# Autodesk Inventor assembly: Full Scale Assembly
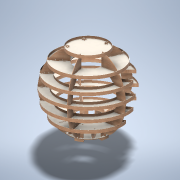
[picture p0: Inventor's stored thumbnail of the model, 180x180]
Saved by Autodesk Inventor 2021 (Build 250183000, 183)
## iProperties
Created: 2020-05-11
Part Number: Full Scale Assembly
Document SubType Name: Assembly
Designer: Dan Wikman
Author: Dan Wikman
## Documents named in this file (34)
- C:\Users\danny\OneDrive\University Life\2020, Semester 1\METR4900 Honours Thesis\Full Scale Design\Full Scale Assembly.iam
- C:\Users\danny\OneDrive\University Life\2020, Semester 1\METR4900 Honours Thesis\Full Scale Design\Disk A.ipt
- C:\Users\danny\OneDrive\University Life\2020, Semester 1\METR4900 Honours Thesis\Full Scale Design\Support A Assembly Dual.iam
- C:\Users\danny\OneDrive\University Life\2020, Semester 1\METR4900 Honours Thesis\Full Scale Design\Support A Assembly Single RIGHT.iam
- C:\Users\danny\OneDrive\University Life\2020, Semester 1\METR4900 Honours Thesis\Full Scale Design\Support A Assembly Single LEFT.iam
- C:\Users\danny\OneDrive\University Life\2020, Semester 1\METR4900 Honours Thesis\Full Scale Design\Support A1.ipt
- C:\Users\danny\OneDrive\University Life\2020, Semester 1\METR4900 Honours Thesis\Full Scale Design\Disc B Assembly.iam
- C:\Users\danny\OneDrive\University Life\2020, Semester 1\METR4900 Honours Thesis\Full Scale Design\Support B.ipt
- C:\Users\danny\OneDrive\University Life\2020, Semester 1\METR4900 Honours Thesis\Full Scale Design\Disc C Assembly.iam
- C:\Users\danny\OneDrive\University Life\2020, Semester 1\METR4900 Honours Thesis\Full Scale Design\Support C.ipt
- C:\Users\danny\OneDrive\University Life\2020, Semester 1\METR4900 Honours Thesis\Full Scale Design\Disk D Assembly.iam
- C:\Users\danny\OneDrive\University Life\2020, Semester 1\METR4900 Honours Thesis\Full Scale Design\Support D.ipt
- C:\Users\danny\OneDrive\University Life\2020, Semester 1\METR4900 Honours Thesis\Full Scale Design\Disc E Assembly.iam
- C:\Users\danny\OneDrive\University Life\2020, Semester 1\METR4900 Honours Thesis\Full Scale Design\Support E.ipt
- C:\Users\danny\OneDrive\University Life\2020, Semester 1\METR4900 Honours Thesis\Full Scale Design\Disk F Assembly.iam
- C:\Users\danny\OneDrive\University Life\2020, Semester 1\METR4900 Honours Thesis\Full Scale Design\Support F.ipt
- C:\Users\danny\OneDrive\University Life\2020, Semester 1\METR4900 Honours Thesis\Full Scale Design\Disk G.ipt
- C:\Users\danny\OneDrive\University Life\2020, Semester 1\METR4900 Honours Thesis\Full Scale Design\Wedge Dual Assembly.iam
- C:\Users\danny\OneDrive\University Life\2020, Semester 1\METR4900 Honours Thesis\Full Scale Design\Feet.ipt
- C:\Users\danny\OneDrive\University Life\2020, Semester 1\METR4900 Honours Thesis\Full Scale Design\Edge Band - Disk G.ipt
- C:\Users\danny\OneDrive\University Life\2020, Semester 1\METR4900 Honours Thesis\Full Scale Design\Edge Band - Platform F Outer.ipt
- C:\Users\danny\OneDrive\University Life\2020, Semester 1\METR4900 Honours Thesis\Full Scale Design\Edge Band - Platform E Inner.ipt
- C:\Users\danny\OneDrive\University Life\2020, Semester 1\METR4900 Honours Thesis\Full Scale Design\Edge Band - Platform E Outer.ipt
- C:\Users\danny\OneDrive\University Life\2020, Semester 1\METR4900 Honours Thesis\Full Scale Design\Edge Band - Platform D Inner.ipt
- C:\Users\danny\OneDrive\University Life\2020, Semester 1\METR4900 Honours Thesis\Full Scale Design\Edge Band - Platform D Outer.ipt
- C:\Users\danny\OneDrive\University Life\2020, Semester 1\METR4900 Honours Thesis\Full Scale Design\Edge Band - Platform C Inner.ipt
- C:\Users\danny\OneDrive\University Life\2020, Semester 1\METR4900 Honours Thesis\Full Scale Design\Edge Band - Platform C Outer.ipt
- C:\Users\danny\OneDrive\University Life\2020, Semester 1\METR4900 Honours Thesis\Full Scale Design\Edge Band - Platform B Outer.ipt
- C:\Users\danny\OneDrive\University Life\2020, Semester 1\METR4900 Honours Thesis\Full Scale Design\Edge Band - Disk A.ipt
- C:\Users\danny\OneDrive\University Life\2020, Semester 1\METR4900 Honours Thesis\Full Scale Design\Edge Band - Platform E Flat.ipt
- C:\Users\danny\OneDrive\University Life\2020, Semester 1\METR4900 Honours Thesis\Full Scale Design\Edge Band - Platform D Flat.ipt
- C:\Users\danny\OneDrive\University Life\2020, Semester 1\METR4900 Honours Thesis\Full Scale Design\Edge Band - Platform C Flat.ipt
- C:\Users\danny\OneDrive\University Life\2020, Semester 1\METR4900 Honours Thesis\Full Scale Design\Edge Band - Platform B Flat.ipt
- C:\Users\danny\OneDrive\University Life\2020, Semester 1\METR4900 Honours Thesis\Full Scale Design\Edge Band - Disk A Inner.ipt
## Components (90 placed, 33 different names)
1. Disk A:1 — Mate:1, Mate:2, Mate:3, Mate:4, Mate:6, Mate:7, Mate:8, Mate:9, Mate:10, Mate:11, Mate:12, Mate:13, Mate:14, Mate:45, Mate:47, Mate:68
2. Support A Assembly Single RIGHT:1 [sub-assembly] — Mate:6, Mate:7, Mate:8
3. Support A Assembly Single LEFT:1 [sub-assembly] — Mate:9, Mate:10, Mate:11, Flush:1, Mate:19, Mate:46, Flush:7, Mate:67
4. Disc B Assembly:1 [sub-assembly] — Mate:15, Mate:16, Mate:17, Mate:18, Mate:66, Flush:13, Mate:81, Mate:82, Mate:83, Mate:85
5. Disc C Assembly:1 [sub-assembly] — Mate:20, Mate:21, Mate:22, Mate:23, Mate:62, Mate:64, Mate:77, Mate:79
6. Disk D Assembly:1 [sub-assembly] — Mate:25, Mate:26, Mate:27, Mate:28, Mate:59, Flush:10, Mate:60, Flush:12, Mate:73, Mate:75
7. Disc E Assembly:1 [sub-assembly] — Mate:30, Mate:31, Mate:32, Mate:33, Mate:55, Flush:8, Mate:57, Flush:9, Mate:69, Mate:71
8. Disk F Assembly:1 [sub-assembly] — Mate:35, Mate:36, Mate:37, Mate:38, Mate:53
9. Disk G:1 — Mate:40, Mate:41, Mate:42, Mate:43, Mate:51
10. Edge Band - Disk G:1 — Mate:50, Mate:51
11. Edge Band - Platform F Outer:1 — Mate:52, Mate:53
12. Edge Band - Platform E Inner:1 — Mate:54, Mate:55, Flush:8
13. Edge Band - Platform E Outer:1 — Mate:56, Mate:57, Flush:9, Flush:14, Mate:70, Flush:15, Mate:72
14. Edge Band - Platform D Inner:1 — Mate:58, Mate:59, Flush:10, Flush:11
15. Edge Band - Platform D Outer:1 — Flush:11, Mate:60, Flush:12, Flush:16, Mate:74, Flush:17, Mate:76
16. Edge Band - Platform C Inner:1 — Mate:61, Mate:62
17. Edge Band - Platform C Outer:1 — Mate:63, Mate:64, Flush:18, Mate:78, Flush:19, Mate:80
18. Edge Band - Platform B Outer:1 — Mate:65, Mate:66, Flush:13, Flush:20, Flush:21, Mate:84, Flush:22
19. Edge Band - Disk A:1 — Mate:67, Mate:68
20. Edge Band - Platform E Flat:1 — Mate:69, Flush:14, Mate:70
21. Edge Band - Platform E Flat:2 — Mate:71, Flush:15, Mate:72
22. Edge Band - Platform D Flat:1 — Mate:73, Flush:16, Mate:74
23. Edge Band - Platform D Flat:2 — Mate:75, Flush:17, Mate:76
24. Edge Band - Platform C Flat:1 — Mate:77, Flush:18, Mate:78
25. Edge Band - Platform C Flat:2 — Mate:79, Flush:19, Mate:80
26. Edge Band - Platform B Flat:1 — Mate:83, Flush:21, Mate:84
27. Edge Band - Platform B Flat:2 — Mate:81, Mate:82, Flush:20
28. Edge Band - Disk A Inner:1 — Flush:22, Mate:85
29. Support A Assembly Dual:1 [sub-assembly] — Mate:1, Mate:2, Mate:3, Mate:49
30. Support A Assembly Dual:2 [sub-assembly] — Mate:16, Mate:17
31. Support A Assembly Dual:3 [sub-assembly]
32. Support A1:1 — Mate:12, Mate:13, Mate:14
33. Support A1:2
34. Support A1:3
35. Support A1:4 — Mate:15
36. Support B:1 — Mate:18, Flush:1, Mate:19, Flush:2, Mate:24, Mate:61, Mate:65
37. Support B:2
38. Support B:3
39. Support B:4 — Mate:20, Mate:21, Mate:22
40. Support B:5
41. Support C:1 — Mate:23, Flush:2, Mate:24, Flush:3, Mate:29, Mate:63
42. Support C:2
43. Support C:3
44. Support C:4 — Mate:25, Mate:26, Mate:27
45. Support C:5
46. Support D:1 — Mate:28, Flush:3, Mate:29, Flush:4, Mate:34, Mate:56, Mate:58
47. Support D:2
48. Support D:3
49. Support D:4 — Mate:30, Mate:31, Mate:32
50. Support D:5
51. Support E:1 — Mate:33, Flush:4, Mate:34, Flush:5, Mate:39
52. Support E:2 — Mate:52
53. Support E:3
54. Support E:4 — Mate:35, Mate:36, Mate:37
55. Support E:5 — Mate:54
56. Support F:1 — Mate:38, Flush:5, Mate:39, Mate:50
57. Support F:2 — Mate:40
58. Support F:3
59. Support F:4 — Mate:41, Mate:42
60. Support F:5 — Mate:44, Flush:6
61. Wedge Dual Assembly:1 [sub-assembly] — Mate:43, Mate:44, Flush:6
62. Wedge Dual Assembly:2 [sub-assembly]
63. Wedge Dual Assembly:3 [sub-assembly]
64. Wedge Dual Assembly:4 [sub-assembly]
65. Wedge Dual Assembly:5 [sub-assembly]
66. Wedge Dual Assembly:6 [sub-assembly] — Mate:45, Mate:46, Flush:7
67. Wedge Dual Assembly:7 [sub-assembly]
68. Wedge Dual Assembly:8 [sub-assembly]
69. Wedge Dual Assembly:9 [sub-assembly]
70. Wedge Dual Assembly:10 [sub-assembly] — Mate:48
71. Feet:1 — Mate:47, Mate:48, Mate:49
72. Feet:2
73. Feet:3
74. Feet:4
75. Feet:5
76. Feet:6
77. Feet:7
78. Feet:8
79. Feet:9
80. Feet:10
81. Feet:11
82. Feet:12
83. Feet:13
84. Feet:14
85. Feet:15
86. Feet:16
87. Feet:17
88. Feet:18
89. Feet:19
90. Feet:20
## Component patterns: (3 elements, first: Support A Assembly Dual:1), (4 elements, first: Support A1:1), (5 elements, first: Support B:1), (5 elements, first: Support C:1), (5 elements, first: Support D:1), (5 elements, first: Support E:1), (5 elements, first: Support F:1), (5 elements, first: Wedge Dual Assembly:1), (5 elements, first: Wedge Dual Assembly:6), (5 elements), (4 elements, first: Feet:1), Component Pattern 10:2 (4 elements), Component Pattern 10:3 (4 elements), Component Pattern 10:4 (4 elements), Component Pattern 10:5 (4 elements)
## Relationships (106: Mate 84, Flush 22)
- Mate:1: Disk A:1 ↔ Support A Assembly Dual:1
- Mate:2 (4 mm): Disk A:1 ↔ Support A Assembly Dual:1
- Mate:3 (0.5 mm): Disk A:1 ↔ Support A Assembly Dual:1
- Mate:4: Disk A:1
- Mate:6: Disk A:1 ↔ Support A Assembly Single RIGHT:1
- Mate:7 (0.5 mm): Disk A:1 ↔ Support A Assembly Single RIGHT:1
- Mate:8 (4 mm): Disk A:1 ↔ Support A Assembly Single RIGHT:1
- Mate:9 (0.5 mm): Disk A:1 ↔ Support A Assembly Single LEFT:1
- Mate:10: Disk A:1 ↔ Support A Assembly Single LEFT:1
- Mate:11 (4 mm): Disk A:1 ↔ Support A Assembly Single LEFT:1
- Mate:12 (0.5 mm): Disk A:1 ↔ Support A1:1
- Mate:13: Disk A:1 ↔ Support A1:1
- Mate:14 (4 mm): Disk A:1 ↔ Support A1:1
- Mate:15: Disc B Assembly:1 ↔ Support A1:4
- Mate:16 (24 mm): Disc B Assembly:1 ↔ Support A Assembly Dual:2
- Mate:17 (0.5 mm): Disc B Assembly:1 ↔ Support A Assembly Dual:2
- Mate:18: Disc B Assembly:1 ↔ Support B:1
- Flush:1: Support A Assembly Single LEFT:1 ↔ Support B:1
- Mate:19 (0.75 mm): Support A Assembly Single LEFT:1 ↔ Support B:1
- Mate:20: Disc C Assembly:1 ↔ Support B:4
- Mate:21 (0.5 mm): Disc C Assembly:1 ↔ Support B:4
- Mate:22 (24 mm): Disc C Assembly:1 ↔ Support B:4
- Mate:23: Disc C Assembly:1 ↔ Support C:1
- Flush:2: Support B:1 ↔ Support C:1
- Mate:24 (1.5 mm): Support B:1 ↔ Support C:1
- Mate:25: Disk D Assembly:1 ↔ Support C:4
- Mate:26 (24 mm): Disk D Assembly:1 ↔ Support C:4
- Mate:27 (0.5 mm): Disk D Assembly:1 ↔ Support C:4
- Mate:28: Disk D Assembly:1 ↔ Support D:1
- Flush:3: Support C:1 ↔ Support D:1
- Mate:29 (1.5 mm): Support C:1 ↔ Support D:1
- Mate:30: Disc E Assembly:1 ↔ Support D:4
- Mate:31 (0.5 mm): Disc E Assembly:1 ↔ Support D:4
- Mate:32 (24 mm): Disc E Assembly:1 ↔ Support D:4
- Mate:33: Disc E Assembly:1 ↔ Support E:1
- Flush:4: Support D:1 ↔ Support E:1
- Mate:34 (1.5 mm): Support D:1 ↔ Support E:1
- Mate:35: Disk F Assembly:1 ↔ Support E:4
- Mate:36 (0.5 mm): Disk F Assembly:1 ↔ Support E:4
- Mate:37 (24 mm): Disk F Assembly:1 ↔ Support E:4
- Mate:38: Disk F Assembly:1 ↔ Support F:1
- Flush:5: Support E:1 ↔ Support F:1
- Mate:39 (1.5 mm): Support E:1 ↔ Support F:1
- Mate:40: Disk G:1 ↔ Support F:2
- Mate:41 (0.5 mm): Disk G:1 ↔ Support F:4
- Mate:42 (4 mm): Disk G:1 ↔ Support F:4
- Mate:43: Disk G:1 ↔ Wedge Dual Assembly:1
- Mate:44 (0.5 mm): Support F:5 ↔ Wedge Dual Assembly:1
- Flush:6 (-51 mm): Support F:5 ↔ Wedge Dual Assembly:1
- Mate:45: Disk A:1 ↔ Wedge Dual Assembly:6
- Mate:46 (0.5 mm): Support A Assembly Single LEFT:1 ↔ Wedge Dual Assembly:6
- Flush:7 (-51 mm): Support A Assembly Single LEFT:1 ↔ Wedge Dual Assembly:6
- Mate:47: Disk A:1 ↔ Feet:1
- Mate:48 (0.5 mm): Wedge Dual Assembly:10 ↔ Feet:1
- Mate:49 (0.5 mm): Support A Assembly Dual:1 ↔ Feet:1
- Mate:50: Edge Band - Disk G:1 ↔ Support F:1
- Mate:51: Disk G:1 ↔ Edge Band - Disk G:1
- Mate:52: Edge Band - Platform F Outer:1 ↔ Support E:2
- Mate:53: Disk F Assembly:1 ↔ Edge Band - Platform F Outer:1
- Mate:54: Edge Band - Platform E Inner:1 ↔ Support E:5
- Mate:55: Disc E Assembly:1 ↔ Edge Band - Platform E Inner:1
- Flush:8: Disc E Assembly:1 ↔ Edge Band - Platform E Inner:1
- Mate:56: Edge Band - Platform E Outer:1 ↔ Support D:1
- Mate:57: Disc E Assembly:1 ↔ Edge Band - Platform E Outer:1
- Flush:9: Disc E Assembly:1 ↔ Edge Band - Platform E Outer:1
- Mate:58: Edge Band - Platform D Inner:1 ↔ Support D:1
- Mate:59: Disk D Assembly:1 ↔ Edge Band - Platform D Inner:1
- Flush:10: Disk D Assembly:1 ↔ Edge Band - Platform D Inner:1
- Flush:11: Edge Band - Platform D Inner:1 ↔ Edge Band - Platform D Outer:1
- Mate:60: Disk D Assembly:1 ↔ Edge Band - Platform D Outer:1
- Flush:12: Disk D Assembly:1 ↔ Edge Band - Platform D Outer:1
- Mate:61: Edge Band - Platform C Inner:1 ↔ Support B:1
- Mate:62: Disc C Assembly:1 ↔ Edge Band - Platform C Inner:1
- Mate:63: Edge Band - Platform C Outer:1 ↔ Support C:1
- Mate:64: Disc C Assembly:1 ↔ Edge Band - Platform C Outer:1
- Mate:65: Edge Band - Platform B Outer:1 ↔ Support B:1
- Mate:66: Disc B Assembly:1 ↔ Edge Band - Platform B Outer:1
- Flush:13: Disc B Assembly:1 ↔ Edge Band - Platform B Outer:1
- Mate:67: Support A Assembly Single LEFT:1 ↔ Edge Band - Disk A:1
- Mate:68: Disk A:1 ↔ Edge Band - Disk A:1
- Mate:69: Disc E Assembly:1 ↔ Edge Band - Platform E Flat:1
- Flush:14: Edge Band - Platform E Outer:1 ↔ Edge Band - Platform E Flat:1
- Mate:70: Edge Band - Platform E Outer:1 ↔ Edge Band - Platform E Flat:1
- Mate:71: Disc E Assembly:1 ↔ Edge Band - Platform E Flat:2
- Flush:15: Edge Band - Platform E Outer:1 ↔ Edge Band - Platform E Flat:2
- Mate:72: Edge Band - Platform E Outer:1 ↔ Edge Band - Platform E Flat:2
- Mate:73: Disk D Assembly:1 ↔ Edge Band - Platform D Flat:1
- Flush:16: Edge Band - Platform D Outer:1 ↔ Edge Band - Platform D Flat:1
- Mate:74: Edge Band - Platform D Outer:1 ↔ Edge Band - Platform D Flat:1
- Mate:75: Disk D Assembly:1 ↔ Edge Band - Platform D Flat:2
- Flush:17: Edge Band - Platform D Outer:1 ↔ Edge Band - Platform D Flat:2
- Mate:76: Edge Band - Platform D Outer:1 ↔ Edge Band - Platform D Flat:2
- Mate:77: Disc C Assembly:1 ↔ Edge Band - Platform C Flat:1
- Flush:18: Edge Band - Platform C Outer:1 ↔ Edge Band - Platform C Flat:1
- Mate:78: Edge Band - Platform C Outer:1 ↔ Edge Band - Platform C Flat:1
- Mate:79: Disc C Assembly:1 ↔ Edge Band - Platform C Flat:2
- Flush:19: Edge Band - Platform C Outer:1 ↔ Edge Band - Platform C Flat:2
- Mate:80: Edge Band - Platform C Outer:1 ↔ Edge Band - Platform C Flat:2
- Mate:81: Disc B Assembly:1 ↔ Edge Band - Platform B Flat:2
- Mate:82: Disc B Assembly:1 ↔ Edge Band - Platform B Flat:2
- Flush:20: Edge Band - Platform B Outer:1 ↔ Edge Band - Platform B Flat:2
- Mate:83: Disc B Assembly:1 ↔ Edge Band - Platform B Flat:1
- Flush:21: Edge Band - Platform B Outer:1 ↔ Edge Band - Platform B Flat:1
- Mate:84: Edge Band - Platform B Outer:1 ↔ Edge Band - Platform B Flat:1
- Flush:22: Edge Band - Platform B Outer:1 ↔ Edge Band - Disk A Inner:1
- Mate:85: Disc B Assembly:1 ↔ Edge Band - Disk A Inner:1
